# Autodesk Inventor assembly: 36-Tooth Differential Assembly
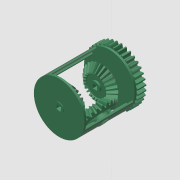
[picture p0: Inventor's stored thumbnail of the model, 180x180]
Saved by Autodesk Inventor 2020 (Build 240168000, 168)
## iProperties
Document SubType Name: Assembly
Designer: Jordan Kiesel
Description: Create more efficient "car style" drivetrains.
Vendor: VEX Robotics, Inc.
Catalog Web Link: vexrobotics.com/276-2184.html
Created: 2019-05-18
Part Number: 36-Tooth Differential Assembly
Category: Motion
Company: Super Sonic Sparks, Team 24
Translation Standard: STEP AP203
FileName: 36-tooth Differential Assembly.iam
PreProcessor: SolidWorks 2006052
PostProcessor: Build: 239, Release: 2011 RTM - Date: Wed 02/17/2010
Sent Units: inch
Uncertainty: 1e-05
Author: Jordan Kiesel
Title: 36-tooth Differential Assembly
Comments: This can be utilized to create more efficient "car style" drivetrains.
## Documents named in this file (3)
- C:\Users\aresp\Documents\Vault\常用部件库\vex原厂部件\36-Tooth Differential Assembly.iam
- C:\Users\aresp\Documents\Inventor\Content Center Files\R2020\zh-CN\24-Tooth Bevel Gear\24-tooth Bevel Gear (2015).ipt
- C:\Users\aresp\Documents\Inventor\Content Center Files\R2020\zh-CN\36-Tooth Differential Housing\Acetal Resin, Dark Sea Green.ipt
## Components (4 placed, 2 different names)
1. 24-Tooth Bevel Gear 24-tooth Bevel Gear (2015):1
2. 36-Tooth Differential Housing Acetal Resin, Dark Sea Green:1
3. 24-Tooth Bevel Gear 24-tooth Bevel Gear (2015):2
4. 24-Tooth Bevel Gear 24-tooth Bevel Gear (2015):3
## Relationships (5: Insert 3, RelateRotation 2)
- [Insert]: 24-Tooth Bevel Gear 24-tooth Bevel Gear (2015):1 ↔ 36-Tooth Differential Housing Acetal Resin, Dark Sea Green:1
- [Insert]: 36-Tooth Differential Housing Acetal Resin, Dark Sea Green:1 ↔ 24-Tooth Bevel Gear 24-tooth Bevel Gear (2015):2
- [Insert]: 36-Tooth Differential Housing Acetal Resin, Dark Sea Green:1 ↔ 24-Tooth Bevel Gear 24-tooth Bevel Gear (2015):3
- [RelateRotation] (1 ul): 24-Tooth Bevel Gear 24-tooth Bevel Gear (2015):1 ↔ 24-Tooth Bevel Gear 24-tooth Bevel Gear (2015):3
- [RelateRotation] (1 ul): 24-Tooth Bevel Gear 24-tooth Bevel Gear (2015):2 ↔ 24-Tooth Bevel Gear 24-tooth Bevel Gear (2015):3
